# Autodesk Inventor assembly: InputShaft
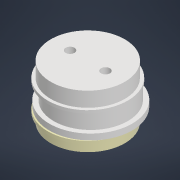
[picture p0: Inventor's stored thumbnail of the model, 180x180]
Saved by Autodesk Inventor 2022 (Build 260153000, 153)
## iProperties
Created: 2022-10-10
Part Number: InputShaft
Document SubType Name: Assembly
Designer: MicnedSQ
Author: MicnedSQ
## Documents named in this file (4)
- C:\Users\MicnedSQ\Desktop\RobotArmV1\RotatingBase\CycloidalDrive\InputShaft.iam
- C:\Users\MicnedSQ\Desktop\RobotArmV1\RotatingBase\CycloidalDrive\InputShaft1.ipt
- C:\Users\MicnedSQ\Desktop\RobotArmV1\RotatingBase\CycloidalDrive\InputShaft2.ipt
- C:\Users\MicnedSQ\Desktop\RobotArmV1\RotatingBase\CycloidalDrive\InputShaft3.ipt
## Components (3 placed, 3 different names)
1. InputShaft1:1 — Rigid:1
2. InputShaft2:1 — Rigid:1, Rigid:2
3. InputShaft3:1 — Rigid:2
## Relationships (2: WeldJoint 2)
- Rigid:1 [WeldJoint]: InputShaft1:1 ↔ InputShaft2:1
- Rigid:2 [WeldJoint]: InputShaft2:1 ↔ InputShaft3:1
